# Autodesk Inventor assembly: Universal Shaft Angle
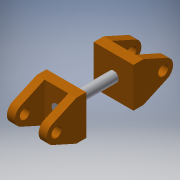
[picture p0: Inventor's stored thumbnail of the model, 180x180]
Saved by Autodesk Inventor 2019 Beta2 (Build 230110000, 110) ContinuousBuild 0
## iProperties
Created: 2014-03-12
Part Number: Universal Shaft Angle
Document SubType Name: Assembly
Designer: John
Author: John
## Documents named in this file (3)
- C:\Users\helfenj\Desktop\Ex_Files_Autodesk_Inventor_2019_EssT\Exercise Files\14_Using constraints to position parts\14_02\Universal Shaft Angle.iam
- C:\Users\helfenj\Desktop\Ex_Files_Autodesk_Inventor_2019_EssT\Exercise Files\14_Using constraints to position parts\14_02\Joint.ipt
- C:\Users\helfenj\Desktop\Ex_Files_Autodesk_Inventor_2019_EssT\Exercise Files\14_Using constraints to position parts\14_02\Connecting Rod.ipt
## Components (3 placed, 2 different names)
1. Joint:3 — Flush:1, Mate:1
2. Connecting Rod:1 — Flush:1, Mate:1, Flush:2, Mate:2
3. Joint:4 — Flush:2, Mate:2
## Relationships (4: Flush 2, Mate 2)
- Flush:1: Joint:3 ↔ Connecting Rod:1
- Mate:1: Joint:3 ↔ Connecting Rod:1
- Flush:2: Connecting Rod:1 ↔ Joint:4
- Mate:2: Connecting Rod:1 ↔ Joint:4
